# Autodesk Inventor assembly: Road_Shaft
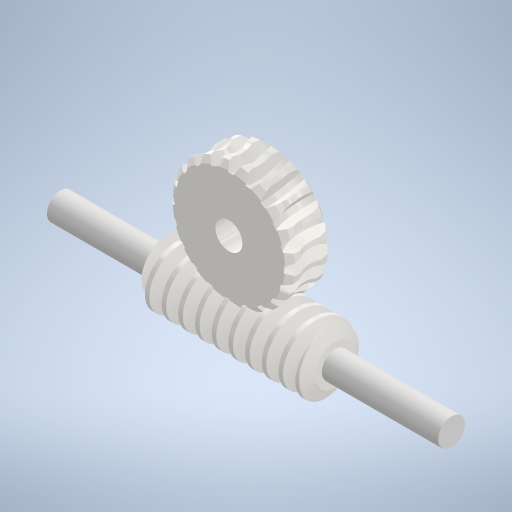
[picture p0: Inventor's stored thumbnail of the model, 512x512]
Saved by Autodesk Inventor 2023 (Build 270158000, 158)
## iProperties
Created: 2023-02-10
Part Number: Road_Shaft
Document SubType Name: Assembly
Designer: deepa
Author: deepa
## Documents named in this file (3)
- C:\Users\deepa\OneDrive\Desktop\Courses\4thsem\ta220\Group 27 TA\Road_Shaft.iam
- C:\Users\deepa\OneDrive\Desktop\Courses\4thsem\ta220\Group 27 TA\shaft temp.ipt
- C:\Users\deepa\OneDrive\Desktop\Courses\4thsem\ta220\Group 27 TA\Road_Shaft\Design Accelerator\Worm Gears7.iam
## Components (2 placed, 2 different names)
1. shaft temp:1 — Mate:3
2. Worm Gears:7 [sub-assembly] — Mate:3
## Relationships (1: Mate 1)
- Mate:3: shaft temp:1 ↔ Worm Gears:7
